# Autodesk Inventor assembly: leg_B_23
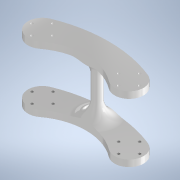
[picture p0: Inventor's stored thumbnail of the model, 180x180]
Saved by Autodesk Inventor 2020.2 (Build 242310000, 310)
## iProperties
Created: 2020-11-22
Part Number: leg_B_23
Document SubType Name: Assembly
Designer: mazzo
Author: mazzo
## Documents named in this file (2)
- D:\Documenti\università\Progetto Meccanica dei Robot\assembled in urdf\leg_B_23.iam
- D:\Documenti\università\Progetto Meccanica dei Robot\meccanica\parti autodesk\V6\V6 Luca\gamba2.ipt
## Components (1 placed, 1 different names)
1. gamba2:1 — Coincidente:1, Coincidente:2, Coincidente:3
## Relationships (3: Mate 3)
- Coincidente:1 [Mate]: gamba2:1
- Coincidente:2 [Mate]: gamba2:1
- Coincidente:3 [Mate]: gamba2:1
